# Autodesk Inventor assembly: Aerogenerador
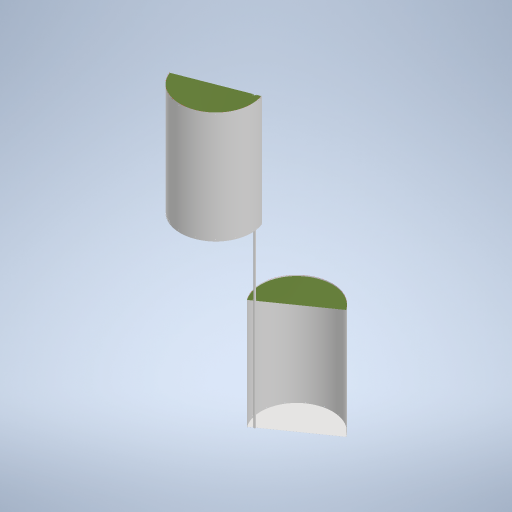
[picture p0: Inventor's stored thumbnail of the model, 512x512]
Saved by Autodesk Inventor 2024 (Build 280153000, 153)
## iProperties
Created: 2024-04-25
Part Number: Aerogenerador
Document SubType Name: Assembly
Designer: alexa
Author: alexa
## Documents named in this file (3)
- C:\Users\alexa\OneDrive\Escritorio\Energia Eolica\Aerogenerador.iam
- C:\Users\alexa\OneDrive\Escritorio\Energia Eolica\Eje.ipt
- C:\Users\alexa\OneDrive\Escritorio\Energia Eolica\Aspa.iam
## Components (3 placed, 2 different names)
1. Eje:1 — Mate:1, Insert:1, Insert:2
2. Aspa:1 [sub-assembly] — Insert:1
3. Aspa:2 [sub-assembly] — Insert:2
## Relationships (3: Insert 2, Mate 1)
- Mate:1: Eje:1
- Insert:1: Eje:1 ↔ Aspa:1
- Insert:2 (-25 mm): Eje:1 ↔ Aspa:2
